# Autodesk Inventor assembly: gear_mirrored
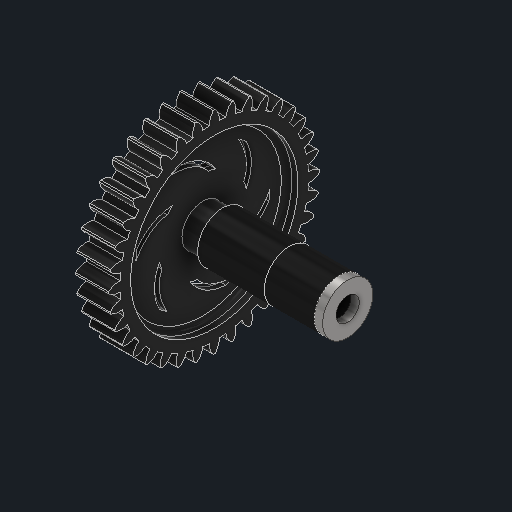
[picture p0: Inventor's stored thumbnail of the model, 512x512]
Saved by Autodesk Inventor 2024 (Build 280153000, 153)
## iProperties
Created: 2024-03-23
Part Number: gear_mirrored
Document SubType Name: Assembly
Designer: Averey Ku
Author: Averey Ku
## Documents named in this file (7)
- D:\vex_robotics\hardware\cad\infection\chassis\mirrored_parts\gear_mirrored.iam
- D:\vex_robotics\hardware\cad\infection\chassis\mirrored_parts\LS 36T Gear_mirrored.ipt
- D:\vex_robotics\hardware\cad\VEX-CAD-Inventor-1.41\Motion\Spacers\Spacer Nylon .375 OD\NSpacer .375 OD x .375.ipt
- D:\vex_robotics\hardware\cad\VEX-CAD-Inventor-1.41\Motion\Spacers\Spacer Nylon .375 OD.ipt
- D:\vex_robotics\hardware\cad\VEX-CAD-Inventor-1.41\Motion\Spacers\Spacer Nylon .375 OD\NSpacer .375 OD x .500.ipt
- D:\vex_robotics\hardware\cad\VEX-CAD-Inventor-1.41\Motion\Spacers\Washer Steel\SWasher .375 OD x .062500.ipt
- D:\vex_robotics\hardware\cad\VEX-CAD-Inventor-1.41\Motion\Spacers\Washer Steel.ipt
## Components (5 placed, 4 different names)
1. LS 36T Gear_mirrored:1 — Insert:4, Insert:2
2. NSpacer .375 OD x .375:1 — Insert:1, Insert:3
3. NSpacer .375 OD x .500:2 — Insert:4, Insert:1
4. SWasher .375 OD x .062500:1 — Insert:3
5. SWasher .375 OD x .062500:2 — Insert:2
## Relationships (4: Insert 4)
- Insert:4: LS 36T Gear_mirrored:1 ↔ NSpacer .375 OD x .500:2
- Insert:1: NSpacer .375 OD x .375:1 ↔ NSpacer .375 OD x .500:2
- Insert:3: NSpacer .375 OD x .375:1 ↔ SWasher .375 OD x .062500:1
- Insert:2: LS 36T Gear_mirrored:1 ↔ SWasher .375 OD x .062500:2
